# Autodesk Inventor assembly: WheelBack
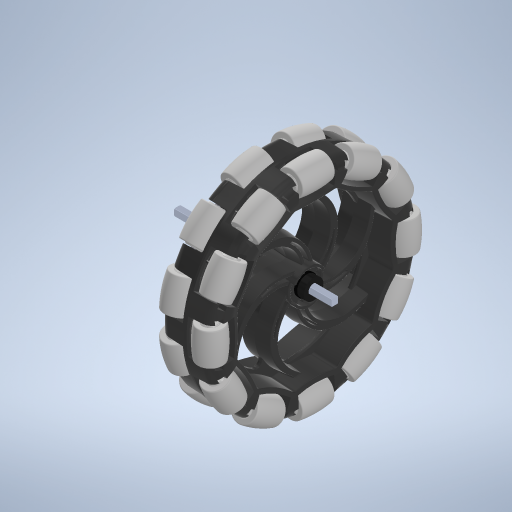
[picture p0: Inventor's stored thumbnail of the model, 512x512]
Saved by Autodesk Inventor 2023 (Build 270158000, 158)
## iProperties
Created: 2022-08-31
Part Number: WheelBack
Document SubType Name: Assembly
Designer: alex
Author: alex
## Documents named in this file (8)
- C:\Users\alex\Documents\GitHub\4067X_spin_up_cad\Chassis\WheelBack.iam
- C:\Users\alex\Documents\GitHub\4067X_spin_up_cad\Library\Motion\Spacers\Spacer Nylon .375 OD\NSpacer .375 OD x .125.ipt
- C:\Users\alex\Documents\GitHub\4067X_spin_up_cad\Library\Motion\Spacers\Spacer Nylon .375 OD.ipt
- C:\Users\alex\Documents\GitHub\4067X_spin_up_cad\Library\Motion\Spacers\Spacer Nylon .375 OD\NSpacer .375 OD x .500.ipt
- C:\Users\alex\Documents\GitHub\4067X_spin_up_cad\Library\Motion\Shaft Collar with Set Screw.ipt
- C:\Users\alex\Documents\GitHub\4067X_spin_up_cad\Library\Motion\Wheels\Omnis\4 Omni, Square.ipt
- C:\Users\alex\Documents\GitHub\4067X_spin_up_cad\Library\Motion\Shaft LS\Shaft LS 3.0 in.ipt
- C:\Users\alex\Documents\GitHub\4067X_spin_up_cad\Library\Motion\Shaft LS.ipt
## Components (6 placed, 5 different names)
1. NSpacer .375 OD x .125:1 — Insert:1, Flush:1
2. Shaft Collar with Set Screw:1 — Insert:1, Insert:6
3. NSpacer .375 OD x .500:2 — Insert:4, Insert:6
4. 4 Omni, Square:1 — Insert:4, Mate:1, Mate:2, Insert:7
5. Shaft LS 3.0 in:1 — Mate:1, Mate:2, Flush:1
6. NSpacer .375 OD x .125:3 — Insert:7
## Relationships (7: Insert 4, Mate 2, Flush 1)
- Insert:1: NSpacer .375 OD x .125:1 ↔ Shaft Collar with Set Screw:1
- Insert:4: NSpacer .375 OD x .500:2 ↔ 4 Omni, Square:1
- Insert:6: Shaft Collar with Set Screw:1 ↔ NSpacer .375 OD x .500:2
- Mate:1: 4 Omni, Square:1 ↔ Shaft LS 3.0 in:1
- Mate:2: 4 Omni, Square:1 ↔ Shaft LS 3.0 in:1
- Flush:1 (24.003 mm): NSpacer .375 OD x .125:1 ↔ Shaft LS 3.0 in:1
- Insert:7: 4 Omni, Square:1 ↔ NSpacer .375 OD x .125:3
